# Autodesk Inventor assembly: Body_Assembly
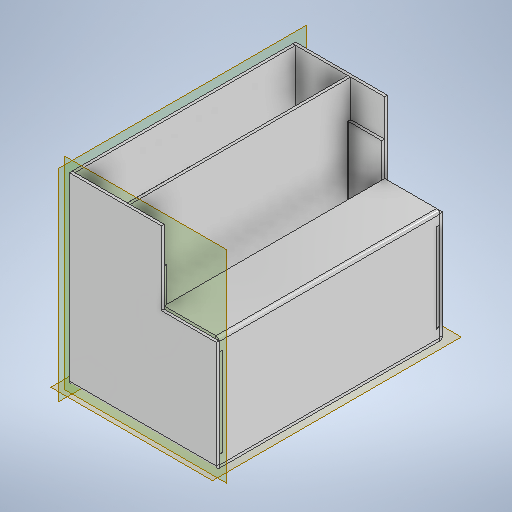
[picture p0: Inventor's stored thumbnail of the model, 512x512]
Saved by Autodesk Inventor 2025.2 (Build 292293000, 293)
## iProperties
Created: 2025-05-07
Part Number: Body_Assembly
Document SubType Name: Assembly
Designer: chris
Author: chris
## Documents named in this file (6)
- C:\Users\chris\문서\Inventor\RHp_Humanoid_ver1\Assembly\1_Body.iam
- C:\Users\chris\문서\Inventor\RHp_Humanoid_ver1\Part\Frame\Body\body_main_frame.ipt
- C:\Users\chris\문서\Inventor\RHp_Humanoid_ver1\Part\Frame\Body\body_front_frame.ipt
- C:\Users\chris\문서\Inventor\RHp_Humanoid_ver1\Part\Frame\Body\body_middle_frame.ipt
- C:\Users\chris\문서\Inventor\RHp_Humanoid_ver1\Part\Frame\Body\body_back_frame.ipt
- C:\Users\chris\문서\Inventor\RHp_Humanoid_ver1\Part\Frame\Body\body_motor_R_frame.ipt
## Components (5 placed, 5 different names)
1. body_main_frame:1 — Mate:1, Mate:2, Mate:3, Mate:4, Flush:1, Mate:5, Mate:6, Flush:3, Mate:7, Mate:8, Flush:4
2. body_front_frame:1 — Mate:1, Mate:2, Mate:3, Flush:2, Mate:9
3. body_middle_frame:1 — Flush:2, Mate:6, Flush:3
4. body_back_frame:1 — Mate:7, Mate:8, Flush:4
5. body_motor_R_frame:1 — Mate:9
## Relationships (13: Mate 9, Flush 4)
- Mate:1: body_main_frame:1 ↔ body_front_frame:1
- Mate:2: body_main_frame:1 ↔ body_front_frame:1
- Mate:3: body_main_frame:1 ↔ body_front_frame:1
- Mate:4: body_main_frame:1
- Flush:1: body_main_frame:1
- Mate:5: body_main_frame:1
- Flush:2 (30 mm): body_front_frame:1 ↔ body_middle_frame:1
- Mate:6: body_main_frame:1 ↔ body_middle_frame:1
- Flush:3: body_main_frame:1 ↔ body_middle_frame:1
- Mate:7: body_main_frame:1 ↔ body_back_frame:1
- Mate:8: body_main_frame:1 ↔ body_back_frame:1
- Flush:4: body_main_frame:1 ↔ body_back_frame:1
- Mate:9: body_front_frame:1 ↔ body_motor_R_frame:1
